# Autodesk Inventor assembly: C-MLG9-75
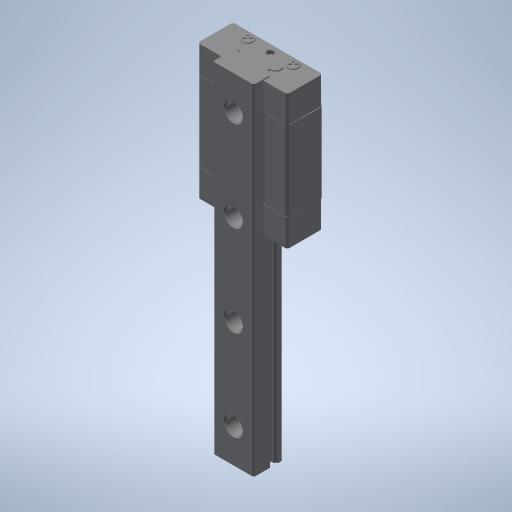
[picture p0: Inventor's stored thumbnail of the model, 512x512]
Saved by Autodesk Inventor 2024.1 (Build 281209000, 209)
## iProperties
Created: 2023-11-06
Part Number: C-MLG9-75
Catalog Web Link: www.cadenas.de
Description: C-MLG, E-GMLG-Economy Miniature Liner Guides - Standard Type
Vendor: MISUMI
Document SubType Name: Assembly
Designer: psAdmin
Manufacturer: MISUMI
Mass: 6.79625 g
Surface Area: 53.2819 cm^2
Volume: 6.79625 cm^3
Density: 1 g/cm^3
Category: PARTsolutions
Company: MISUMI
PSOL_IDENT_0: {$CADENAS_DATA/23d-libs/misumi/metric/06_linear_guides/c_mlg_asmtab.prj},221 {VTYP=3D},{STYP=ASSTAB}
PSOL_IDENT_1: ,{NB=C-MLG9-75},{LINA=C-MLG9-75},{NN=C-MLG, E-GMLG},{DATE=23.08.2023 07:24:55},{GEOMDATE=23.08.2023
PSOL_IDENT_2: 07:24:48},{VERSION=},{LINEID=20},{WBVAR=ST,L,ALT1,ALT2,ALT3,ALT4,ES,ALT5,EB},{WBNUMERIC=L,ES,EB}  {N
PSOL_IDENT_3: B=C-MLG9-75},{LINA=C-MLG9-75},{KT=DUMMY},{PN=C-MLG9-75},{TYPE=C-MLG},{ST=1},{NM=9},{L=75},{LALG=[35:
PSOL_IDENT_4: 900/1]},{H=10},{H1=2.0},{N=5.5},{W=20},{B=15},{B1=2.5},{C=10},{L1=17.5},{L2=29.60},{GNN=Dia.1.4},{MX
PSOL_IDENT_5: L=M3*3},{H2=1.8},{WRR=9},{HRR=6.5},{D=6.0},{HH=3.5},{DD=3.6},{P=20},{M=4},{E=7.5},{ALT1=},{ALT2=},{A
PSOL_IDENT_6: LT3=},{ALT4=},{ES=0.0},{ESALG=0},{ESMIN=2.000},{ESMAX=13.000},{ALT4PN=},{ALT5=},{ALT5ALG='','w/o EB
PSOL_IDENT_7: (Right end face E size specification)','EB','with EB (Right end face E size specification)' },{EB=0.
PSOL_IDENT_8: 0},{EBALG=0},{EBMIN=2.000},{EBMAX=13.000},{ALT5PN=},{PPATH=c_mlg/c_mlg_asmtpl.prj}
NB: C-MLG9-75
NN: C-MLG, E-GMLG
NT: Economy Miniature Liner Guides - Standard Type
NBSYN: $PN.
LINA: C-MLG9-75
CATALOG: Misumi
PN: C-MLG9-75
ST: No Surface Treatment
L: 75
H: 10
H1: 2
N: 5.5
W: 20
B: 15
B1: 2.5
C: 10
L1: 17.5
L2: 29.6
GNN: Dia.1.4
MXL: M3*3
H2: 1.8
WRR: 9
HRR: 6.5
D: 6
HH: 3.5
DD: 3.6
P: 20
E: 7.5
ALT1: w/o MC (Tapped Holes)
ALT2: w/o (Additional Blocks)
ALT3: w/o Z1 (Pressure Change)
ALT4: w/o ES (Left end face E size specification)
ES: 0
ALT5: w/o EB (Right end face E size specification)
EB: 0
SUPPLIER: MISUMI
ARTICLENO: C-MLG9-75
BOMINFO: C-MLG9-75
CREATOR: CADENAS GmbH
Title: C-MLG9-75
Author: Cadenas PARTsolutions
Comments: Economy Miniature Liner Guides - Standard Type
## Documents named in this file (3)
- C:\Users\haruy\OneDrive - Kyushu University\KURT_工房共有\2023~2024\ハード\CAD\2024NHK\000_parts\スライダー\C-MLG9-75_Autodesk_Inventor_2024_20231106 (1)\AIS2024\C-MLG9-75.iam
- C:\Users\haruy\OneDrive - Kyushu University\KURT_工房共有\2023~2024\ハード\CAD\2024NHK\000_parts\スライダー\C-MLG9-75_Autodesk_Inventor_2024_20231106 (1)\AIS2024\C-MLG9-75_r.ipt
- C:\Users\haruy\OneDrive - Kyushu University\KURT_工房共有\2023~2024\ハード\CAD\2024NHK\000_parts\スライダー\C-MLG9-75_Autodesk_Inventor_2024_20231106 (1)\AIS2024\C-MLGB9.ipt
## Components (2 placed, 2 different names)
1. C-MLG9-75_r:1 — to_block1_Z@1 <-> to_rail_Z@2, to_block1_YZ@1 <-> to_rail_YZ@2
2. C-MLGB9:1 — to_block1_Z@1 <-> to_rail_Z@2, to_block1_YZ@1 <-> to_rail_YZ@2
## Relationships (2: Mate 1, Angle 1)
- to_block1_Z@1 <-> to_rail_Z@2 [Mate]: C-MLG9-75_r:1 ↔ C-MLGB9:1
- to_block1_YZ@1 <-> to_rail_YZ@2 [Angle] (0 deg): C-MLG9-75_r:1 ↔ C-MLGB9:1
